# Autodesk Inventor assembly: assembly_test
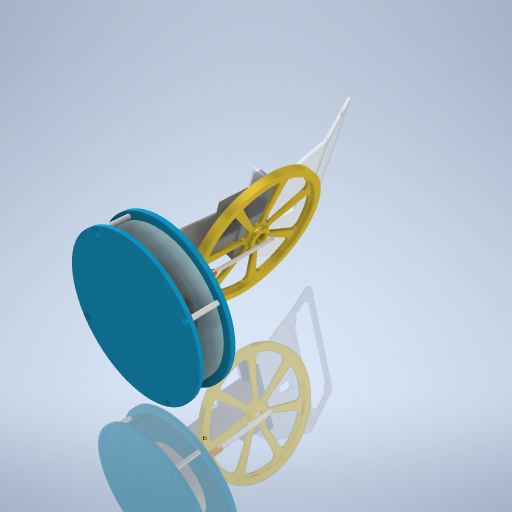
[picture p0: Inventor's stored thumbnail of the model, 512x512]
Saved by Autodesk Inventor 2024.2 (Build 282272000, 272)
## iProperties
Created: 2024-04-06
Part Number: assembly_test
Document SubType Name: Assembly
Designer: Fabri
Author: Fabri
## Documents named in this file (19)
- C:\Users\Fabri\Documents\Inventor\Stirlingmotor\assembly_test.iam
- C:\Users\Fabri\Documents\Inventor\Stirlingmotor\plate.ipt
- C:\Users\Fabri\Documents\Inventor\Stirlingmotor\cylinder.ipt
- C:\Users\Fabri\Documents\Inventor\Stirlingmotor\steuerkolben.ipt
- C:\Users\Fabri\Documents\Inventor\Stirlingmotor\stange.ipt
- C:\Users\Fabri\Documents\Inventor\Stirlingmotor\plate_2.ipt
- C:\Users\Fabri\Documents\Inventor\Stirlingmotor\Lagerbock.ipt
- C:\Users\Fabri\Documents\Inventor\Stirlingmotor\Ak zylinder.ipt
- C:\Users\Fabri\Documents\Inventor\Stirlingmotor\Arbeitskolben.ipt
- C:\Users\Fabri\Documents\Inventor\Stirlingmotor\Gewindehülse.ipt
- C:\Users\Fabri\Documents\Inventor\Stirlingmotor\Führungsbüchse.ipt
- C:\Users\Fabri\Documents\Inventor\Stirlingmotor\kopf.ipt
- C:\Users\Fabri\Documents\Inventor\Stirlingmotor\pleuelstange.ipt
- C:\Users\Fabri\Documents\Inventor\Stirlingmotor\Rad.ipt
- C:\Users\Fabri\Documents\Inventor\Stirlingmotor\Kurbel.ipt
- C:\Users\Fabri\Documents\Inventor\Stirlingmotor\Glaswinkel.ipt
- C:\Users\Fabri\Documents\Inventor\Stirlingmotor\Flach_Alu.ipt
- C:\Users\Fabri\Documents\Inventor\Stirlingmotor\büchse.ipt
- C:\Users\Fabri\Documents\Inventor\Stirlingmotor\kurbelwelle.ipt
## Components (24 placed, 18 different names)
1. plate:1 — Einfügen:1, Passend:1
2. cylinder:1 — Einfügen:1
3. steuerkolben:1 — Einfügen:33
4. plate_2:1 — Einfügen:5, Winkel:1, Einfügen:8, Einfügen:9, Einfügen:10, Einfügen:11
5. Lagerbock:1 — Einfügen:5, Winkel:1, Einfügen:17, Einfügen:18, Fluchtend:1, Einfügen:20, Passend:6
6. Ak zylinder:1 — Zylindrisch:1
7. Arbeitskolben:1 — Einfügen:29, Zylindrisch:1
8. Gewindehülse:1 — Einfügen:11
9. Gewindehülse:2 — Einfügen:8, Passend:2, Passend:3
10. Gewindehülse:3 — Einfügen:9
11. Gewindehülse:4 — Einfügen:10
12. kopf:1 — Einfügen:31, Einfügen:32
13. pleuelstange:1 — Einfügen:26, Winkel:8, Einfügen:31
14. Rad:1 — Passend:5, Einfügen:21, main_motion, Winkel:6, Winkel:7, Einfügen:26, Einfügen:30, Winkel:8
15. pleuelstange:2 — Winkel:7, Einfügen:22, Einfügen:23
16. Kurbel:1 — Einfügen:17, Winkel:6, Einfügen:22
17. Glaswinkel:1 — Einfügen:18, Fluchtend:1, Einfügen:19, Fluchtend:2
18. Flach_Alu:1 — Einfügen:19, Fluchtend:2
19. büchse:1 — Einfügen:20, Einfügen:30
20. kurbelwelle:1 — Einfügen:21
21. kopf:2 — Einfügen:23, Einfügen:24
22. stange:2 — Einfügen:24, Einfügen:29
23. stange:3 — Einfügen:32, Zylindrisch:2, Einfügen:33
24. Führungsbüchse:1 — Zylindrisch:2
## Relationships (35: Insert 20, Mate 6, Angle 5, Flush 2, CylindricalJoint 2)
- Einfügen:1 [Insert]: plate:1 ↔ cylinder:1
- Einfügen:5 [Insert]: plate_2:1 ↔ Lagerbock:1
- Winkel:1 [Angle] (180 deg): plate_2:1 ↔ Lagerbock:1
- Einfügen:8 [Insert] (-19 mm): plate_2:1 ↔ Gewindehülse:2
- Passend:1 [Mate]: plate:1
- Passend:2 [Mate]: Gewindehülse:2
- Passend:3 [Mate]: Gewindehülse:2
- Einfügen:9 [Insert] (-21 mm): plate_2:1 ↔ Gewindehülse:3
- Einfügen:10 [Insert] (-21 mm): plate_2:1 ↔ Gewindehülse:4
- Einfügen:11 [Insert] (-21 mm): plate_2:1 ↔ Gewindehülse:1
- Einfügen:17 [Insert] (-0.9 mm): Lagerbock:1 ↔ Kurbel:1
- Einfügen:18 [Insert]: Lagerbock:1 ↔ Glaswinkel:1
- Fluchtend:1 [Flush]: Lagerbock:1 ↔ Glaswinkel:1
- Einfügen:19 [Insert]: Glaswinkel:1 ↔ Flach_Alu:1
- Fluchtend:2 [Flush]: Glaswinkel:1 ↔ Flach_Alu:1
- Einfügen:20 [Insert] (-15 mm): Lagerbock:1 ↔ büchse:1
- Passend:5 [Mate]: Rad:1
- Passend:6 [Mate]: Lagerbock:1
- Passend:7 [Mate]
- Einfügen:21 [Insert] (-25 mm): Rad:1 ↔ kurbelwelle:1
- main_motion [Angle] (0 deg): Rad:1
- Winkel:6 [Angle] (48.5 deg): Rad:1 ↔ Kurbel:1
- Winkel:7 [Angle] (140 deg): Rad:1 ↔ pleuelstange:2
- Einfügen:22 [Insert] (1.45 mm): pleuelstange:2 ↔ Kurbel:1
- Einfügen:23 [Insert] (0.12 mm): pleuelstange:2 ↔ kopf:2
- Einfügen:24 [Insert] (-5 mm): kopf:2 ↔ stange:2
- Einfügen:26 [Insert] (3.5 mm): pleuelstange:1 ↔ Rad:1
- Einfügen:29 [Insert] (-15 mm): Arbeitskolben:1 ↔ stange:2
- Zylindrisch:1 [CylindricalJoint]: Ak zylinder:1 ↔ Arbeitskolben:1
- Einfügen:30 [Insert] (1.5 mm): Rad:1 ↔ büchse:1
- Winkel:8 [Angle] (0 deg): pleuelstange:1 ↔ Rad:1
- Einfügen:31 [Insert]: kopf:1 ↔ pleuelstange:1
- Einfügen:32 [Insert] (-10.5 mm): kopf:1 ↔ stange:3
- Zylindrisch:2 [CylindricalJoint]: stange:3 ↔ Führungsbüchse:1
- Einfügen:33 [Insert]: steuerkolben:1 ↔ stange:3
